# Autodesk Inventor assembly: zlozenie_v1
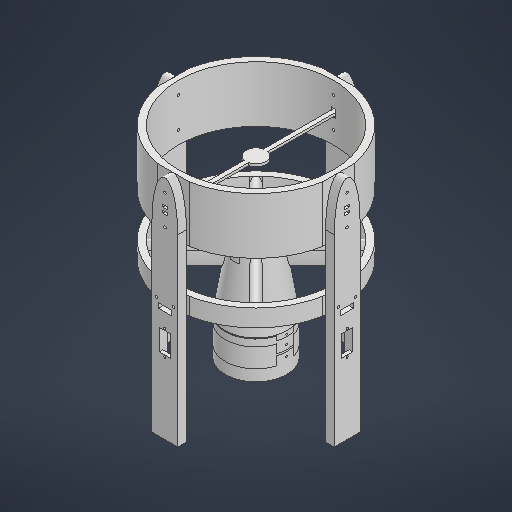
[picture p0: Inventor's stored thumbnail of the model, 512x512]
Saved by Autodesk Inventor 2026 (Build 300175000, 175)
## iProperties
Created: 2026-04-21
Part Number: zlozenie_v1
Document SubType Name: Assembly
Designer: Patryk Lombardo
Author: Patryk Lombardo
## Documents named in this file (8)
- C:\Users\Patryk Lombardo\Desktop\Coaxial\cad\zlozenie_v1.iam
- C:\Users\Patryk Lombardo\Desktop\Coaxial\cad\001-001.ipt
- C:\Users\Patryk Lombardo\Desktop\Coaxial\cad\002-002.ipt
- C:\Users\Patryk Lombardo\Desktop\Coaxial\cad\003-001.ipt
- C:\Users\Patryk Lombardo\Desktop\Coaxial\cad\004-002.ipt
- C:\Users\Patryk Lombardo\Desktop\Coaxial\cad\005-001.ipt
- C:\Users\Patryk Lombardo\Desktop\Coaxial\cad\007-002.ipt
- C:\Users\Patryk Lombardo\Desktop\Coaxial\cad\008-002.ipt
## Components (10 placed, 7 different names)
1. 001-001:1 — Zestawiające:9, Zestawiające:10, Zestawiające:11, Zestawiające:12, Zestawiające:13, Zestawiające:14, Zestawiające:15
2. 002-002:1 — Zestawiające:5, Zestawiające:6, Zestawiające:7, Zestawiające:8
3. 003-001:1 — Zestawiające:3, Zestawiające:4, Zestawiające:5, Zestawiające:6
4. 004-002:1 — Zestawiające:1, Zestawiające:2, Zestawiające:3, Zestawiające:4, Zestawiające:16, Zestawiające:17
5. 005-001:1 — Zestawiające:1, Zestawiające:2
6. 007-002:1 — Zestawiające:7, Zestawiające:8
7. 008-002:1 — Zestawiające:14, Zestawiające:15, Zestawiające:16, Zestawiające:17
8. 008-002:2 — Zestawiające:13
9. 008-002:3 — Zestawiające:11, Zestawiające:12
10. 008-002:4 — Zestawiające:9, Zestawiające:10
## Relationships (17: Mate 17)
- Zestawiające:1 [Mate]: 004-002:1 ↔ 005-001:1
- Zestawiające:2 [Mate]: 004-002:1 ↔ 005-001:1
- Zestawiające:3 [Mate]: 003-001:1 ↔ 004-002:1
- Zestawiające:4 [Mate]: 003-001:1 ↔ 004-002:1
- Zestawiające:5 [Mate]: 002-002:1 ↔ 003-001:1
- Zestawiające:6 [Mate]: 002-002:1 ↔ 003-001:1
- Zestawiające:7 [Mate]: 002-002:1 ↔ 007-002:1
- Zestawiające:8 [Mate]: 002-002:1 ↔ 007-002:1
- Zestawiające:9 [Mate]: 001-001:1 ↔ 008-002:4
- Zestawiające:10 [Mate]: 001-001:1 ↔ 008-002:4
- Zestawiające:11 [Mate]: 001-001:1 ↔ 008-002:3
- Zestawiające:12 [Mate]: 001-001:1 ↔ 008-002:3
- Zestawiające:13 [Mate]: 001-001:1 ↔ 008-002:2
- Zestawiające:14 [Mate]: 001-001:1 ↔ 008-002:1
- Zestawiające:15 [Mate]: 001-001:1 ↔ 008-002:1
- Zestawiające:16 [Mate]: 004-002:1 ↔ 008-002:1
- Zestawiające:17 [Mate]: 004-002:1 ↔ 008-002:1
